# Autodesk Inventor assembly: drillTool1
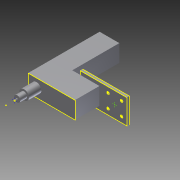
[picture p0: Inventor's stored thumbnail of the model, 180x180]
Saved by Autodesk Inventor 2012 (Build 160160000, 160)
## iProperties
Created: 2012-06-20
Part Number: drillTool1
Document SubType Name: Assembly
Designer: wberry
Author: wberry
## Documents named in this file (3)
- C:\Users\wberry\Documents\MATLAB\plate Calibration\models cad\drillTool_1.iam
- C:\Users\wberry\Documents\MATLAB\plate Calibration\models cad\tool Part1.ipt
- C:\Users\wberry\Documents\MATLAB\plate Calibration\models cad\Part4.ipt
## Components (2 placed, 2 different names)
1. tool Part1:1 — Mate:1, Mate:2, Flush:1
2. Part4:1 — Mate:1, Mate:2, Flush:1
## Relationships (3: Mate 2, Flush 1)
- Mate:1: tool Part1:1 ↔ Part4:1
- Mate:2 (20 mm): tool Part1:1 ↔ Part4:1
- Flush:1 (9.64 mm): tool Part1:1 ↔ Part4:1
